# Autodesk Inventor assembly: сборка акб
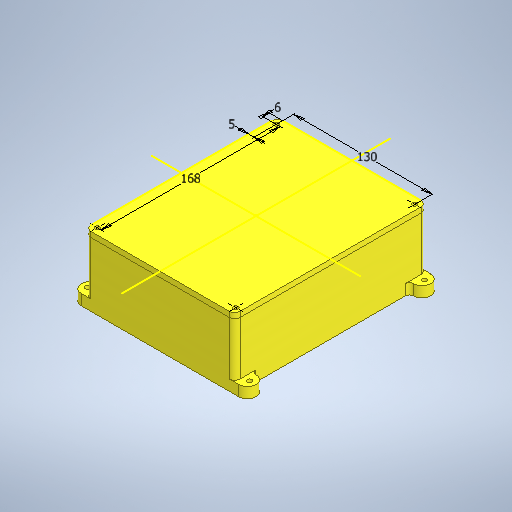
[picture p0: Inventor's stored thumbnail of the model, 512x512]
Saved by Autodesk Inventor 2025 (Build 290162000, 162)
## iProperties
Created: 2025-02-26
Part Number: сборка акб
Document SubType Name: Assembly
Designer: volko
Author: volko
## Documents named in this file (5)
- C:\Users\volko\Desktop\диплом\Модели\детали\сборка акб.iam
- C:\Users\volko\Desktop\диплом\Модели\детали\акб корпус.ipt
- C:\Users\volko\Desktop\диплом\Модели\детали\акб.ipt
- C:\Users\volko\Desktop\диплом\Модели\детали\акб_MIR.ipt
- C:\Users\volko\Desktop\диплом\Модели\детали\крышка акб.ipt
## Components (4 placed, 4 different names)
1. акб корпус:1 — Заподлицо:1, Заподлицо:2, Заподлицо:3, Совмещение:1, Заподлицо:4, Совмещение:2, Совмещение:3, Совмещение:6
2. акб:1 — Совмещение:1, Заподлицо:4, Совмещение:2, Симметрия:1
3. акб_MIR:1 — Симметрия:1, Совмещение:3, Совмещение:4
4. крышка акб:1 — Совмещение:5, Совмещение:6, Заподлицо:5
## Relationships (12: Mate 6, Flush 5, Symmetry 1)
- Заподлицо:1 [Flush]: акб корпус:1
- Заподлицо:2 [Flush]: акб корпус:1
- Заподлицо:3 [Flush]: акб корпус:1
- Совмещение:1 [Mate]: акб корпус:1 ↔ акб:1
- Заподлицо:4 [Flush]: акб корпус:1 ↔ акб:1
- Совмещение:2 [Mate] (3.5 mm): акб корпус:1 ↔ акб:1
- Симметрия:1 [Symmetry]: акб:1 ↔ акб_MIR:1
- Совмещение:3 [Mate]: акб корпус:1 ↔ акб_MIR:1
- Совмещение:4 [Mate]: акб_MIR:1
- Совмещение:5 [Mate]: крышка акб:1
- Совмещение:6 [Mate]: акб корпус:1 ↔ крышка акб:1
- Заподлицо:5 [Flush]: крышка акб:1
